# Autodesk Inventor assembly: Tall Cupboard
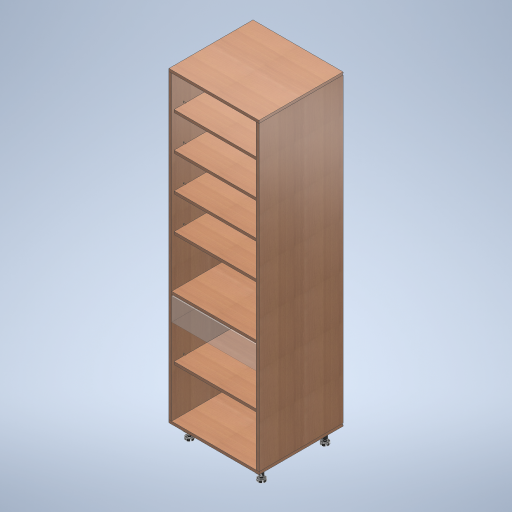
[picture p0: Inventor's stored thumbnail of the model, 512x512]
Saved by Autodesk Inventor 2024 (Build 280153000, 153)
## iProperties
Created: 2017-05-10
Part Number: Tall Cupboard
Document SubType Name: Assembly
Designer: SauliusD
Author: SauliusD
## Documents named in this file (22)
- C:\W4INV 2024 Design\iBOX LIBRARY\Kitchen\Standing Cabinets\Tall Cupboard\Tall Cupboard.iam
- C:\W4INV 2024 Design\iBOX LIBRARY\Kitchen\Standing Cabinets\Tall Cupboard\Right Panel.ipt
- C:\W4INV 2024 Design\iBOX LIBRARY\Kitchen\Standing Cabinets\Tall Cupboard\Top Panel.ipt
- C:\W4INV 2024 Design\iBOX LIBRARY\Kitchen\Standing Cabinets\Tall Cupboard\Left Panel.ipt
- C:\W4INV 2024 Design\iBOX LIBRARY\Kitchen\Standing Cabinets\Tall Cupboard\Bottom Panel.ipt
- C:\W4INV 2024 Design\iBOX LIBRARY\Kitchen\Standing Cabinets\Tall Cupboard\Back Panel.ipt
- C:\W4INV 2024 Design\iBOX LIBRARY\Kitchen\Standing Cabinets\Tall Cupboard\Bottom Shelf.ipt
- C:\W4INV 2024 Design\iBOX LIBRARY\Kitchen\Standing Cabinets\Tall Cupboard\Drawers Space.ipt
- C:\W4INV 2024 Design\iBOX LIBRARY\Kitchen\Standing Cabinets\Tall Cupboard\Horizontal Partition_1.ipt
- C:\W4INV 2024 Design\iBOX LIBRARY\Kitchen\Standing Cabinets\Tall Cupboard\Horizontal Partition1.ipt
- C:\W4INV 2024 Design\_LIBRARY\Fixed joints\Minifix joint\MINIFIX D15 v2\Minifix D15 & Dowel L34 & Cap D15 PB T18 LH.ipt
- C:\W4INV 2024 Design\_LIBRARY\Fixed joints\Confirmat\CONFIRMAT\Confirmat L50 & Cap D10 NB T18 PB T 18.ipt
- C:\W4INV 2024 Design\_LIBRARY\Holders\Shelf holder D5\Shelf support D5 L16 with hole covers.ipt
- C:\W4INV 2024 Design\_LIBRARY\Fixed joints\Minifix joint\MINIFIX D15 v2\Minifix D15 & Dowel L34 & Cap D15 PB T18 RH.ipt
- C:\W4INV 2024 Design\_LIBRARY\Supports and legs\Legs\ADJUSTABLE LEG\Adjustable leg  BT18 clip included.ipt
- C:\W4INV 2024 Design\_LIBRARY\Supports and legs\Legs\ADJUSTABLE LEG\Adjustable leg  BT18.ipt
- C:\W4INV 2024 Design\iBOX LIBRARY\Kitchen\Standing Cabinets\Tall Cupboard\Tall Cupboard.ipt
- C:\W4INV 2024 Design\iBOX LIBRARY\Kitchen\Standing Cabinets\Tall Cupboard\Bottom_shelf.ipt
- C:\W4INV 2023 Design\LIBRARY\Fixed joints\Minifix joint\MINIFIX D15 v2.ipt
- C:\W4INV 2023 Design\LIBRARY\Fixed joints\Confirmat\CONFIRMAT.ipt
- C:\W4INV 2023 Design\LIBRARY\Holders\Shelf holder D5.ipt
- C:\W4INV 2023 Design\LIBRARY\Supports and legs\Legs\ADJUSTABLE LEG.ipt
## Components (50 placed, 17 different names)
1. @Skeleton — Flush:19, Flush:20, Flush:21
2. Right Panel:1 — Flush:1, Flush:2, Pillar Board Side Plane :2, Pillar Board Side Plane :4, Pillar Board Side Plane:2, Pillar Board Side Plane:4, Side Board Plane:4, Side Board Plane:10, Nestled Board Plane:10, Nestled Board Plane:12, Side Board Plane:2, Side Board Plane:6
3. Top Panel:1 — Nestled Board Plane:1, Nestled Board Plane:2, Nestled Board Plane:3, Nestled Board Plane:4
4. Left Panel:1 — Pillar Board Side Plane :1, Pillar Board Side Plane :3, Pillar Board Side Plane:1, Pillar Board Side Plane:3, Side Board Plane:3, Side Board Plane:9, Nestled Board Plane:9, Nestled Board Plane:11, Side Board Plane:5, Side Board Plane:7
5. Bottom Panel:1 — Flush:3, Flush:4, Flush:5, Flush:6, Nestled Board Plane:5, Nestled Board Plane:6, Nestled Board Plane:7, Nestled Board Plane:8, Bottom board Plane:1, Front (Angle) Plane:1, Bottom board Plane:2, Front (Angle) Plane:2, Bottom board Plane:3, Front (Angle) Plane:3, Bottom board Plane:4, Front (Angle) Plane:4
6. Back Panel:1
7. Bottom Shelf:1
8. Drawers Space:1
9. Horizontal Partition_1:1 — Pillar Board Side Plane :5, Pillar Board Side Plane :6, Pillar Board Side Plane :7, Pillar Board Side Plane :8
10. Minifix D15 & Dowel L34 & Cap D15 PB T18 LH:1 — Axis Plane:1, Pillar Board Side Plane :1, Nestled Board Plane:1
11. Minifix D15 & Dowel L34 & Cap D15 PB T18 RH:2 — Axis Plane:2, Pillar Board Side Plane :2, Nestled Board Plane:2
12. Minifix D15 & Dowel L34 & Cap D15 PB T18 RH:3 — Axis Plane:3, Pillar Board Side Plane :3, Nestled Board Plane:3
13. Minifix D15 & Dowel L34 & Cap D15 PB T18 LH:4 — Axis Plane:4, Pillar Board Side Plane :4, Nestled Board Plane:4
14. Confirmat L50 & Cap D10 NB T18 PB T 18:1 — Axis Plane:5, Pillar Board Side Plane:1, Nestled Board Plane:5
15. Confirmat L50 & Cap D10 NB T18 PB T 18:2 — Axis Plane:6, Pillar Board Side Plane:2, Nestled Board Plane:6
16. Confirmat L50 & Cap D10 NB T18 PB T 18:3 — Axis Plane:7, Pillar Board Side Plane:3, Nestled Board Plane:7
17. Confirmat L50 & Cap D10 NB T18 PB T 18:4 — Axis Plane:8, Pillar Board Side Plane:4, Nestled Board Plane:8
18. Minifix D15 & Dowel L34 & Cap D15 PB T18 RH:5 — Axis Plane:21, Nestled Board Plane:9, Pillar Board Side Plane :5
19. Minifix D15 & Dowel L34 & Cap D15 PB T18 LH:6 — Axis Plane:22, Nestled Board Plane:10, Pillar Board Side Plane :6
20. Minifix D15 & Dowel L34 & Cap D15 PB T18 LH:7 — Axis Plane:23, Nestled Board Plane:11, Pillar Board Side Plane :7
21. Minifix D15 & Dowel L34 & Cap D15 PB T18 RH:8 — Axis Plane:24, Nestled Board Plane:12, Pillar Board Side Plane :8
22. Adjustable leg  BT18 clip included:1 — Axis2 Plane:1, Axis Plane:25, Bottom board Plane:1, Front (Angle) Plane:1
23. Adjustable leg  BT18:2 — Axis2 Plane:2, Axis Plane:26, Bottom board Plane:2, Front (Angle) Plane:2
24. Adjustable leg  BT18 clip included:3 — Axis2 Plane:3, Axis Plane:27, Bottom board Plane:3, Front (Angle) Plane:3
25. Adjustable leg  BT18:4 — Axis2 Plane:4, Axis Plane:28, Bottom board Plane:4, Front (Angle) Plane:4
26. Bottom_shelf:1 — Shelf Pottom Plane:1, Shelf Pottom Plane:2, Shelf Pottom Plane:5, Shelf Pottom Plane:6
27. Shelf support D5 L16 with hole covers:24 — Axis Plane:9, Side Board Plane:2, Shelf Pottom Plane:1
28. Shelf support D5 L16 with hole covers:25 — Axis Plane:10, Side Board Plane:5, Shelf Pottom Plane:2
29. Shelf support D5 L16 with hole covers:26 — Axis Plane:13, Side Board Plane:6, Shelf Pottom Plane:5
30. Shelf support D5 L16 with hole covers:27 — Axis Plane:14, Side Board Plane:7, Shelf Pottom Plane:6
31. Horizontal Partition1:1 — Shelf Pottom Plane:3, Shelf Pottom Plane:4, Shelf Pottom Plane:9, Shelf Pottom Plane:10
32. Shelf support D5 L16 with hole covers:10 — Axis Plane:18, Shelf Pottom Plane:10, Side Board Plane:10
33. Shelf support D5 L16 with hole covers:4 — Axis Plane:12, Shelf Pottom Plane:4, Side Board Plane:4
34. Shelf support D5 L16 with hole covers:3 — Axis Plane:11, Shelf Pottom Plane:3, Side Board Plane:3
35. Shelf support D5 L16 with hole covers:9 — Axis Plane:17, Shelf Pottom Plane:9, Side Board Plane:9
36. Horizontal Partition1:2
37. Shelf support D5 L16 with hole covers:11
38. Shelf support D5 L16 with hole covers:12
39. Shelf support D5 L16 with hole covers:13
40. Shelf support D5 L16 with hole covers:14
41. Horizontal Partition1:3
42. Shelf support D5 L16 with hole covers:15
43. Shelf support D5 L16 with hole covers:16
44. Shelf support D5 L16 with hole covers:17
45. Shelf support D5 L16 with hole covers:18
46. Horizontal Partition1:4
47. Shelf support D5 L16 with hole covers:19
48. Shelf support D5 L16 with hole covers:20
49. Shelf support D5 L16 with hole covers:21
50. Shelf support D5 L16 with hole covers:22
## Component patterns: (4 elements, first: Horizontal Partition1:1 + Shelf support D5 L16 with hole covers:10 + Shelf support D5 L16 with hole covers:4 + Shelf support D5 L16 with hole covers:3 + Shelf support D5 L16 with hole covers:9)
## Relationships (85: Mate 60, Flush 21, Angle 4)
- Flush:1 (-80 mm): Right Panel:1
- Flush:2 (-80 mm): Right Panel:1
- Flush:3 (-77 mm): Bottom Panel:1
- Flush:4 (-60 mm): Bottom Panel:1
- Flush:5 (-60 mm): Bottom Panel:1
- Flush:6 (-60 mm): Bottom Panel:1
- Axis Plane:1 [Mate]: Minifix D15 & Dowel L34 & Cap D15 PB T18 LH:1
- Pillar Board Side Plane :1 [Flush] (18 mm): Left Panel:1 ↔ Minifix D15 & Dowel L34 & Cap D15 PB T18 LH:1
- Nestled Board Plane:1 [Mate]: Top Panel:1 ↔ Minifix D15 & Dowel L34 & Cap D15 PB T18 LH:1
- Axis Plane:2 [Mate]: Minifix D15 & Dowel L34 & Cap D15 PB T18 RH:2
- Pillar Board Side Plane :2 [Flush] (18 mm): Right Panel:1 ↔ Minifix D15 & Dowel L34 & Cap D15 PB T18 RH:2
- Nestled Board Plane:2 [Mate]: Top Panel:1 ↔ Minifix D15 & Dowel L34 & Cap D15 PB T18 RH:2
- Axis Plane:3 [Mate]: Minifix D15 & Dowel L34 & Cap D15 PB T18 RH:3
- Pillar Board Side Plane :3 [Flush] (18 mm): Left Panel:1 ↔ Minifix D15 & Dowel L34 & Cap D15 PB T18 RH:3
- Nestled Board Plane:3 [Mate]: Top Panel:1 ↔ Minifix D15 & Dowel L34 & Cap D15 PB T18 RH:3
- Axis Plane:4 [Mate]: Minifix D15 & Dowel L34 & Cap D15 PB T18 LH:4
- Pillar Board Side Plane :4 [Flush] (18 mm): Right Panel:1 ↔ Minifix D15 & Dowel L34 & Cap D15 PB T18 LH:4
- Nestled Board Plane:4 [Mate]: Top Panel:1 ↔ Minifix D15 & Dowel L34 & Cap D15 PB T18 LH:4
- Axis Plane:5 [Mate]: Confirmat L50 & Cap D10 NB T18 PB T 18:1
- Pillar Board Side Plane:1 [Mate] (-9 mm): Left Panel:1 ↔ Confirmat L50 & Cap D10 NB T18 PB T 18:1
- Nestled Board Plane:5 [Flush]: Bottom Panel:1 ↔ Confirmat L50 & Cap D10 NB T18 PB T 18:1
- Axis Plane:6 [Mate]: Confirmat L50 & Cap D10 NB T18 PB T 18:2
- Pillar Board Side Plane:2 [Mate] (-9 mm): Right Panel:1 ↔ Confirmat L50 & Cap D10 NB T18 PB T 18:2
- Nestled Board Plane:6 [Flush]: Bottom Panel:1 ↔ Confirmat L50 & Cap D10 NB T18 PB T 18:2
- Axis Plane:7 [Mate]: Confirmat L50 & Cap D10 NB T18 PB T 18:3
- Pillar Board Side Plane:3 [Mate] (-9 mm): Left Panel:1 ↔ Confirmat L50 & Cap D10 NB T18 PB T 18:3
- Nestled Board Plane:7 [Flush]: Bottom Panel:1 ↔ Confirmat L50 & Cap D10 NB T18 PB T 18:3
- Axis Plane:8 [Mate]: Confirmat L50 & Cap D10 NB T18 PB T 18:4
- Pillar Board Side Plane:4 [Mate] (-9 mm): Right Panel:1 ↔ Confirmat L50 & Cap D10 NB T18 PB T 18:4
- Nestled Board Plane:8 [Flush]: Bottom Panel:1 ↔ Confirmat L50 & Cap D10 NB T18 PB T 18:4
- Axis Plane:11 [Mate]: Shelf support D5 L16 with hole covers:3
- Shelf Pottom Plane:3 [Mate] (2.5 mm): Horizontal Partition1:1 ↔ Shelf support D5 L16 with hole covers:3
- Side Board Plane:3 [Mate]: Left Panel:1 ↔ Shelf support D5 L16 with hole covers:3
- Axis Plane:12 [Mate]: Shelf support D5 L16 with hole covers:4
- Shelf Pottom Plane:4 [Mate] (2.5 mm): Horizontal Partition1:1 ↔ Shelf support D5 L16 with hole covers:4
- Side Board Plane:4 [Mate]: Right Panel:1 ↔ Shelf support D5 L16 with hole covers:4
- Axis Plane:17 [Mate]: Shelf support D5 L16 with hole covers:9
- Shelf Pottom Plane:9 [Mate] (2.5 mm): Horizontal Partition1:1 ↔ Shelf support D5 L16 with hole covers:9
- Side Board Plane:9 [Mate]: Left Panel:1 ↔ Shelf support D5 L16 with hole covers:9
- Axis Plane:18 [Mate]: Shelf support D5 L16 with hole covers:10
- Shelf Pottom Plane:10 [Mate] (2.5 mm): Horizontal Partition1:1 ↔ Shelf support D5 L16 with hole covers:10
- Side Board Plane:10 [Mate]: Right Panel:1 ↔ Shelf support D5 L16 with hole covers:10
- Axis Plane:21 [Mate]: Minifix D15 & Dowel L34 & Cap D15 PB T18 RH:5
- Nestled Board Plane:9 [Mate]: Left Panel:1 ↔ Minifix D15 & Dowel L34 & Cap D15 PB T18 RH:5
- Pillar Board Side Plane :5 [Flush] (18 mm): Horizontal Partition_1:1 ↔ Minifix D15 & Dowel L34 & Cap D15 PB T18 RH:5
- Axis Plane:22 [Mate]: Minifix D15 & Dowel L34 & Cap D15 PB T18 LH:6
- Nestled Board Plane:10 [Mate]: Right Panel:1 ↔ Minifix D15 & Dowel L34 & Cap D15 PB T18 LH:6
- Pillar Board Side Plane :6 [Flush] (18 mm): Horizontal Partition_1:1 ↔ Minifix D15 & Dowel L34 & Cap D15 PB T18 LH:6
- Axis Plane:23 [Mate]: Minifix D15 & Dowel L34 & Cap D15 PB T18 LH:7
- Nestled Board Plane:11 [Mate]: Left Panel:1 ↔ Minifix D15 & Dowel L34 & Cap D15 PB T18 LH:7
- Pillar Board Side Plane :7 [Flush] (18 mm): Horizontal Partition_1:1 ↔ Minifix D15 & Dowel L34 & Cap D15 PB T18 LH:7
- Axis Plane:24 [Mate]: Minifix D15 & Dowel L34 & Cap D15 PB T18 RH:8
- Nestled Board Plane:12 [Mate]: Right Panel:1 ↔ Minifix D15 & Dowel L34 & Cap D15 PB T18 RH:8
- Pillar Board Side Plane :8 [Flush] (18 mm): Horizontal Partition_1:1 ↔ Minifix D15 & Dowel L34 & Cap D15 PB T18 RH:8
- Axis2 Plane:1 [Mate]: Adjustable leg  BT18 clip included:1
- Axis Plane:25 [Mate]: Adjustable leg  BT18 clip included:1
- Bottom board Plane:1 [Mate]: Bottom Panel:1 ↔ Adjustable leg  BT18 clip included:1
- Front (Angle) Plane:1 [Angle] (0 deg): Bottom Panel:1 ↔ Adjustable leg  BT18 clip included:1
- Axis2 Plane:2 [Mate]: Adjustable leg  BT18:2
- Axis Plane:26 [Mate]: Adjustable leg  BT18:2
- Bottom board Plane:2 [Mate]: Bottom Panel:1 ↔ Adjustable leg  BT18:2
- Front (Angle) Plane:2 [Angle] (0 deg): Bottom Panel:1 ↔ Adjustable leg  BT18:2
- Axis2 Plane:3 [Mate]: Adjustable leg  BT18 clip included:3
- Axis Plane:27 [Mate]: Adjustable leg  BT18 clip included:3
- Bottom board Plane:3 [Mate]: Bottom Panel:1 ↔ Adjustable leg  BT18 clip included:3
- Front (Angle) Plane:3 [Angle] (0 deg): Bottom Panel:1 ↔ Adjustable leg  BT18 clip included:3
- Axis2 Plane:4 [Mate]: Adjustable leg  BT18:4
- Axis Plane:28 [Mate]: Adjustable leg  BT18:4
- Bottom board Plane:4 [Mate]: Bottom Panel:1 ↔ Adjustable leg  BT18:4
- Front (Angle) Plane:4 [Angle] (0 deg): Bottom Panel:1 ↔ Adjustable leg  BT18:4
- Flush:19: @Skeleton
- Flush:20: @Skeleton
- Flush:21: @Skeleton
- Axis Plane:9 [Mate]: Shelf support D5 L16 with hole covers:24
- Side Board Plane:2 [Mate]: Right Panel:1 ↔ Shelf support D5 L16 with hole covers:24
- Shelf Pottom Plane:1 [Mate] (2.5 mm): Bottom_shelf:1 ↔ Shelf support D5 L16 with hole covers:24
- Axis Plane:10 [Mate]: Shelf support D5 L16 with hole covers:25
- Side Board Plane:5 [Mate]: Left Panel:1 ↔ Shelf support D5 L16 with hole covers:25
- Shelf Pottom Plane:2 [Mate] (2.5 mm): Bottom_shelf:1 ↔ Shelf support D5 L16 with hole covers:25
- Axis Plane:13 [Mate]: Shelf support D5 L16 with hole covers:26
- Side Board Plane:6 [Mate]: Right Panel:1 ↔ Shelf support D5 L16 with hole covers:26
- Shelf Pottom Plane:5 [Mate] (2.5 mm): Bottom_shelf:1 ↔ Shelf support D5 L16 with hole covers:26
- Axis Plane:14 [Mate]: Shelf support D5 L16 with hole covers:27
- Side Board Plane:7 [Mate]: Left Panel:1 ↔ Shelf support D5 L16 with hole covers:27
- Shelf Pottom Plane:6 [Mate] (2.5 mm): Bottom_shelf:1 ↔ Shelf support D5 L16 with hole covers:27
## Named parameters: Top_Shelf_Qauntity = 3, SpaceBetweenUperShelf = 234.75 mm, Top_Shelfs_Quantity = 3, Top_Shelves_Start_Position = 320 mm, Space_For_Drawer = 160 mm, Bottom_Shelf_Start_Position = 320 mm, Cupboard_Line_Height = 750 mm
